# Autodesk Inventor assembly: Gearboxes_001_assembly for 3
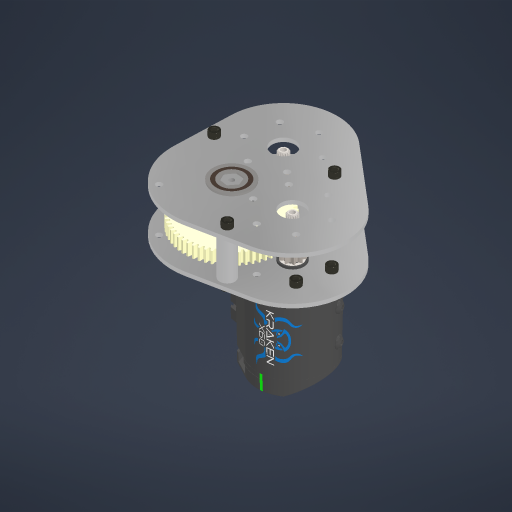
[picture p0: Inventor's stored thumbnail of the model, 512x512]
Saved by Autodesk Inventor 2024.4 (Build 284460000, 460)
## iProperties
Created: 2026-06-11
Part Number: Gearboxes_001_assembly for 3
Document SubType Name: Assembly
Designer: stanr
Author: stanr
## Documents named in this file (10)
- C:\Users\stanr\Documents\GitHub\2026-2027-DesignTraining\Stan\Gearboxes_001_assembly for 3.iam
- C:\Users\stanr\Documents\GitHub\2026-2027-DesignTraining\Stan\Gearboxes_3_thingy that holds motors and more.ipt
- C:\Users\stanr\Documents\GitHub\2026-2027-DesignTraining\COTS Library\Motors\COTS_WCP-0940_KrakenX60_New.ipt
- C:\Users\stanr\Documents\GitHub\2026-2027-DesignTraining\COTS Library\Motion\Bearings\COTS_WCP-0783_1.125ODHexBearing.ipt
- C:\Users\stanr\Documents\GitHub\2026-2027-DesignTraining\Stan\Gearboxes_003_standoff.ipt
- C:\Users\stanr\Documents\GitHub\2026-2027-DesignTraining\Stan\WCP-0720\WCP-0720.ipt
- C:\Users\stanr\Documents\GitHub\2026-2027-DesignTraining\Stan\WCP-0973\WCP-0973.ipt
- C:\Users\stanr\Documents\GitHub\2026-2027-DesignTraining\Stan\WCP-1008\WCP-1008\WCP-1008.ipt
- C:\Users\stanr\Documents\GitHub\2026-2027-DesignTraining\Stan\Gearboxes_002_Hexshaft my fav.ipt
- C:\Users\stanr\Documents\GitHub\2026-2027-DesignTraining\COTS Library\Fasteners\Bolts\Socket-Head\10-32\COTS_91251A342_1-2in Long_Black-Oxide Alloy Steel Socket Head.ipt
## Components (25 placed, 9 different names)
1. Gearboxes_3_thingy that holds motors and more:1 — Mate:65, Mate:66, Mate:67, Mate:68, Mate:69, Mate:70, Mate:71, Mate:72, Mate:73, Mate:78, Mate:79, Mate:80, Mate:81, Mate:82, Mate:90, Mate:91, Mate:92, Mate:93, Mate:94, Mate:95, Mate:97, Mate:99, Mate:100, Mate:101, Mate:103, Mate:107, Mate:108, Mate:109
2. COTS_WCP-0940_KrakenX60_New:1 — Mate:19, Mate:20, Mate:67, Mate:68, Mate:71
3. COTS_WCP-0940_KrakenX60_New:2 — Mate:17, Mate:18, Mate:65, Mate:66, Mate:69, Mate:70
4. Gearboxes_003_standoff:1 — Mate:78, Mate:82, Mate:84, Mate:85, Mate:88
5. Gearboxes_003_standoff:4 — Mate:79, Mate:89, Mate:96, Mate:97
6. WCP-0720:1 — Mate:26, Mate:28, Mate:76, Mate:77
7. WCP-0973:1 — Mate:27, Mate:28
8. WCP-1008:1 — Mate:17, Mate:18
9. WCP-1008:2 — Mate:19, Mate:20
10. Gearboxes_002_Hexshaft my fav:2 — Mate:26, Mate:27, Mate:74, Mate:75, Mate:76, Mate:83
11. COTS_91251A342_1-2in Long_Black-Oxide Alloy Steel Socket Head:1 — Mate:89, Mate:98
12. COTS_91251A342_1-2in Long_Black-Oxide Alloy Steel Socket Head:2 — Mate:94, Mate:99
13. COTS_91251A342_1-2in Long_Black-Oxide Alloy Steel Socket Head:3 — Mate:95, Mate:100
14. COTS_91251A342_1-2in Long_Black-Oxide Alloy Steel Socket Head:5 — Mate:90, Mate:109
15. COTS_91251A342_1-2in Long_Black-Oxide Alloy Steel Socket Head:8 — Mate:87, Mate:105
16. COTS_91251A342_1-2in Long_Black-Oxide Alloy Steel Socket Head:9 — Mate:92, Mate:107
17. COTS_91251A342_1-2in Long_Black-Oxide Alloy Steel Socket Head:11 — Mate:96, Mate:103
18. COTS_91251A342_1-2in Long_Black-Oxide Alloy Steel Socket Head:12 — Mate:93, Mate:101
19. COTS_91251A342_1-2in Long_Black-Oxide Alloy Steel Socket Head:13 — Mate:91, Mate:108
20. COTS_91251A342_1-2in Long_Black-Oxide Alloy Steel Socket Head:15
21. COTS_91251A342_1-2in Long_Black-Oxide Alloy Steel Socket Head:16 — Mate:88, Mate:106
22. COTS_WCP-0783_1.125ODHexBearing:2 — Mate:72, Mate:73, Mate:74, Mate:75, Mate:77
23. COTS_WCP-0783_1.125ODHexBearing:3 — Mate:83, Mate:104
24. Gearboxes_003_standoff:5 — Mate:80, Mate:81, Mate:86, Mate:87
25. Gearboxes_3_thingy that holds motors and more:2 — Mate:84, Mate:85, Mate:86, Mate:98, Mate:104, Mate:105, Mate:106
## Relationships (51: Mate 51)
- Mate:17: COTS_WCP-0940_KrakenX60_New:2 ↔ WCP-1008:1
- Mate:18: COTS_WCP-0940_KrakenX60_New:2 ↔ WCP-1008:1
- Mate:19: COTS_WCP-0940_KrakenX60_New:1 ↔ WCP-1008:2
- Mate:20: COTS_WCP-0940_KrakenX60_New:1 ↔ WCP-1008:2
- Mate:26: WCP-0720:1 ↔ Gearboxes_002_Hexshaft my fav:2
- Mate:27: WCP-0973:1 ↔ Gearboxes_002_Hexshaft my fav:2
- Mate:28: WCP-0720:1 ↔ WCP-0973:1
- Mate:65: Gearboxes_3_thingy that holds motors and more:1 ↔ COTS_WCP-0940_KrakenX60_New:2
- Mate:66: Gearboxes_3_thingy that holds motors and more:1 ↔ COTS_WCP-0940_KrakenX60_New:2
- Mate:67: Gearboxes_3_thingy that holds motors and more:1 ↔ COTS_WCP-0940_KrakenX60_New:1
- Mate:68: Gearboxes_3_thingy that holds motors and more:1 ↔ COTS_WCP-0940_KrakenX60_New:1
- Mate:69: Gearboxes_3_thingy that holds motors and more:1 ↔ COTS_WCP-0940_KrakenX60_New:2
- Mate:70: Gearboxes_3_thingy that holds motors and more:1 ↔ COTS_WCP-0940_KrakenX60_New:2
- Mate:71: Gearboxes_3_thingy that holds motors and more:1 ↔ COTS_WCP-0940_KrakenX60_New:1
- Mate:72: Gearboxes_3_thingy that holds motors and more:1 ↔ COTS_WCP-0783_1.125ODHexBearing:2
- Mate:73: Gearboxes_3_thingy that holds motors and more:1 ↔ COTS_WCP-0783_1.125ODHexBearing:2
- Mate:74: Gearboxes_002_Hexshaft my fav:2 ↔ COTS_WCP-0783_1.125ODHexBearing:2
- Mate:75: Gearboxes_002_Hexshaft my fav:2 ↔ COTS_WCP-0783_1.125ODHexBearing:2
- Mate:76: WCP-0720:1 ↔ Gearboxes_002_Hexshaft my fav:2
- Mate:77: WCP-0720:1 ↔ COTS_WCP-0783_1.125ODHexBearing:2
- Mate:78: Gearboxes_3_thingy that holds motors and more:1 ↔ Gearboxes_003_standoff:1
- Mate:79: Gearboxes_3_thingy that holds motors and more:1 ↔ Gearboxes_003_standoff:4
- Mate:80: Gearboxes_3_thingy that holds motors and more:1 ↔ Gearboxes_003_standoff:5
- Mate:81: Gearboxes_3_thingy that holds motors and more:1 ↔ Gearboxes_003_standoff:5
- Mate:82: Gearboxes_3_thingy that holds motors and more:1 ↔ Gearboxes_003_standoff:1
- Mate:83: Gearboxes_002_Hexshaft my fav:2 ↔ COTS_WCP-0783_1.125ODHexBearing:3
- Mate:84: Gearboxes_003_standoff:1 ↔ Gearboxes_3_thingy that holds motors and more:2
- Mate:85: Gearboxes_003_standoff:1 ↔ Gearboxes_3_thingy that holds motors and more:2
- Mate:86: Gearboxes_003_standoff:5 ↔ Gearboxes_3_thingy that holds motors and more:2
- Mate:87: COTS_91251A342_1-2in Long_Black-Oxide Alloy Steel Socket Head:8 ↔ Gearboxes_003_standoff:5
- Mate:88: Gearboxes_003_standoff:1 ↔ COTS_91251A342_1-2in Long_Black-Oxide Alloy Steel Socket Head:16
- Mate:89: Gearboxes_003_standoff:4 ↔ COTS_91251A342_1-2in Long_Black-Oxide Alloy Steel Socket Head:1
- Mate:90: Gearboxes_3_thingy that holds motors and more:1 ↔ COTS_91251A342_1-2in Long_Black-Oxide Alloy Steel Socket Head:5
- Mate:91: Gearboxes_3_thingy that holds motors and more:1 ↔ COTS_91251A342_1-2in Long_Black-Oxide Alloy Steel Socket Head:13
- Mate:92: Gearboxes_3_thingy that holds motors and more:1 ↔ COTS_91251A342_1-2in Long_Black-Oxide Alloy Steel Socket Head:9
- Mate:93: Gearboxes_3_thingy that holds motors and more:1 ↔ COTS_91251A342_1-2in Long_Black-Oxide Alloy Steel Socket Head:12
- Mate:94: Gearboxes_3_thingy that holds motors and more:1 ↔ COTS_91251A342_1-2in Long_Black-Oxide Alloy Steel Socket Head:2
- Mate:95: Gearboxes_3_thingy that holds motors and more:1 ↔ COTS_91251A342_1-2in Long_Black-Oxide Alloy Steel Socket Head:3
- Mate:96: Gearboxes_003_standoff:4 ↔ COTS_91251A342_1-2in Long_Black-Oxide Alloy Steel Socket Head:11
- Mate:97: Gearboxes_3_thingy that holds motors and more:1 ↔ Gearboxes_003_standoff:4
- Mate:98: COTS_91251A342_1-2in Long_Black-Oxide Alloy Steel Socket Head:1 ↔ Gearboxes_3_thingy that holds motors and more:2
- Mate:99: Gearboxes_3_thingy that holds motors and more:1 ↔ COTS_91251A342_1-2in Long_Black-Oxide Alloy Steel Socket Head:2
- Mate:100: Gearboxes_3_thingy that holds motors and more:1 ↔ COTS_91251A342_1-2in Long_Black-Oxide Alloy Steel Socket Head:3
- Mate:101: Gearboxes_3_thingy that holds motors and more:1 ↔ COTS_91251A342_1-2in Long_Black-Oxide Alloy Steel Socket Head:12
- Mate:103: Gearboxes_3_thingy that holds motors and more:1 ↔ COTS_91251A342_1-2in Long_Black-Oxide Alloy Steel Socket Head:11
- Mate:104: COTS_WCP-0783_1.125ODHexBearing:3 ↔ Gearboxes_3_thingy that holds motors and more:2
- Mate:105: COTS_91251A342_1-2in Long_Black-Oxide Alloy Steel Socket Head:8 ↔ Gearboxes_3_thingy that holds motors and more:2
- Mate:106: COTS_91251A342_1-2in Long_Black-Oxide Alloy Steel Socket Head:16 ↔ Gearboxes_3_thingy that holds motors and more:2
- Mate:107: Gearboxes_3_thingy that holds motors and more:1 ↔ COTS_91251A342_1-2in Long_Black-Oxide Alloy Steel Socket Head:9
- Mate:108: Gearboxes_3_thingy that holds motors and more:1 ↔ COTS_91251A342_1-2in Long_Black-Oxide Alloy Steel Socket Head:13
- Mate:109: Gearboxes_3_thingy that holds motors and more:1 ↔ COTS_91251A342_1-2in Long_Black-Oxide Alloy Steel Socket Head:5
